# Autodesk Inventor assembly: Nanotube Output Cluster
Saved by Autodesk Inventor 2013 (Build 170138000, 138)
## iProperties
Created: 2013-09-01
Part Number: Nanotube Output Cluster
Document SubType Name: Assembly
Designer: Nemo
Mass: 173.205 g
Surface Area: 250.782 cm^2
Volume: 55.1057 cm^3
Density: 3.14314 g/cm^3
Author: Nemo
## Documents named in this file (5)
- H:\Nemo\Documents\Robotics\COTS Parts\Gearboxes\Components\Nanotube Output Cluster.iam
- H:\Nemo\Documents\Robotics\COTS Parts\Gears - VexPro\Gear 20dp 500hex 50T Vex.ipt
- H:\Nemo\Documents\Robotics\COTS Parts\Bearings - VexPro\Flanged Bearing - 0.5in Hex ID x 1.125in OD.ipt
- H:\Nemo\Documents\Robotics\COTS Parts\Bearings - VexPro\Flanged Bearing - 0.5in Round ID x 1.125in OD.ipt
- H:\Nemo\Documents\Robotics\COTS Parts\Gearboxes\Components\AndyMark Shafts\Supershifter Long Hex Output Shaft.ipt
## Components (4 placed, 4 different names)
1. Gear 20dp 500hex 50T Vex:1
2. Flanged Bearing - 0.5in Hex ID x 1.125in OD:1
3. Flanged Bearing - 0.5in Round ID x 1.125in OD:1
4. Supershifter Long Hex Output Shaft:1
## Relationships (2: Mate 1, Insert 1)
- [Mate] (0.254 mm): Gear 20dp 500hex 50T Vex:1 ↔ Flanged Bearing - 0.5in Hex ID x 1.125in OD:1
- [Insert]: Flanged Bearing - 0.5in Round ID x 1.125in OD:1 ↔ Supershifter Long Hex Output Shaft:1
